# Autodesk Inventor assembly: Omniscope_new_v0
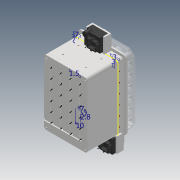
[picture p0: Inventor's stored thumbnail of the model, 180x180]
Saved by Autodesk Inventor 2022 (Build 260153000, 153)
## iProperties
Created: 2022-05-25
Part Number: Omniscope_new_v0
Document SubType Name: Assembly
Designer: diederichbenedict
Author: diederichbenedict
## Documents named in this file (13)
- C:\Users\diederichbenedict\Dropbox\Dokumente\Promotion\PROJECTS\Omniscope\INVENTOR\Omniscope_new_v0.iam
- C:\Users\diederichbenedict\Dropbox\Dokumente\Promotion\PROJECTS\Omniscope\INVENTOR\00_MicroSDCard.ipt
- C:\Users\diederichbenedict\Dropbox\Dokumente\Promotion\PROJECTS\Omniscope\INVENTOR\Omniscope_Base_v0.ipt
- C:\Users\diederichbenedict\Dropbox\Dokumente\Promotion\PROJECTS\Omniscope\INVENTOR\Omniscope_sidewalls_v0.ipt
- C:\Users\diederichbenedict\Dropbox\Dokumente\Promotion\PROJECTS\Omniscope\INVENTOR\Omniscope_mid_level_v0.ipt
- C:\Users\diederichbenedict\Dropbox\Dokumente\Promotion\PROJECTS\Omniscope\INVENTOR\OV_Camera.ipt
- C:\Users\diederichbenedict\Dropbox\Dokumente\Promotion\PROJECTS\Omniscope\INVENTOR\00_ESP3-CAMboard.iam
- C:\Users\diederichbenedict\Dropbox\Dokumente\Promotion\PROJECTS\Omniscope\INVENTOR\Omniscope_Camera_fix.ipt
- C:\Users\diederichbenedict\Dropbox\Dokumente\Promotion\PROJECTS\Omniscope\INVENTOR\00_24wellplate_base.ipt
- C:\Users\diederichbenedict\Dropbox\Dokumente\Promotion\PROJECTS\Omniscope\INVENTOR\Omniscope_sidewall_spacer_v0.ipt
- C:\Users\diederichbenedict\Dropbox\Dokumente\Promotion\PROJECTS\Omniscope\INVENTOR\Omniscope_lensmount_v0.ipt
- C:\Users\diederichbenedict\Dropbox\Dokumente\Promotion\PROJECTS\Omniscope\INVENTOR\00_Z_Focus_CCTV_Camera.ipt
- C:\Users\diederichbenedict\Dropbox\Dokumente\Promotion\PROJECTS\Omniscope\INVENTOR\Omniscope_Wellcarrier.ipt
## Components (106 placed, 12 different names)
1. Omniscope_Base_v0:1 — Passend:1, Passend:2, Passend:3, Fluchtend:3, Fluchtend:4
2. Omniscope_sidewalls_v0:1 — Fluchtend:3, Fluchtend:4, Einfügen:1, Einfügen:2, Passend:7, Fluchtend:7, Fluchtend:8, Fluchtend:15, Fluchtend:16, Passend:8, Passend:9, Passend:10, Fluchtend:17
3. Omniscope_mid_level_v0:1 — Einfügen:1, Einfügen:2, Passend:4, Winkel:1, Passend:5, Passend:6, Fluchtend:5, Fluchtend:6, Fluchtend:9
4. 00_24wellplate_base:1 — Passend:7, Fluchtend:7
5. Omniscope_sidewall_spacer_v0:1 — Fluchtend:8, Fluchtend:9, Fluchtend:10, Fluchtend:11
6. Omniscope_lensmount_v0:1 — Fluchtend:10, Fluchtend:11, Fluchtend:18, Fluchtend:19, Fluchtend:20
7. 00_Z_Focus_CCTV_Camera:1 — Fluchtend:13, Fluchtend:14, Fluchtend:15, Passend:9
8. 00_Z_Focus_CCTV_Camera:2 — Fluchtend:14, Fluchtend:16, Passend:8, Fluchtend:18
9. 00_Z_Focus_CCTV_Camera:3 — Fluchtend:13, Passend:10, Fluchtend:17
10. Omniscope_Wellcarrier:1 — Fluchtend:19, Fluchtend:20
11. 00_MicroSDCard:1 — Passend:1, Passend:2, Fluchtend:1, Fluchtend:2
12. 00_ESP3-CAMboard:1 — Fluchtend:1, Fluchtend:2, Passend:3
13. 00_MicroSDCard:2
14. 00_ESP3-CAMboard:2
15. 00_MicroSDCard:3
16. 00_ESP3-CAMboard:3
17. 00_MicroSDCard:4
18. 00_ESP3-CAMboard:4
19. 00_MicroSDCard:5
20. 00_ESP3-CAMboard:5
21. 00_MicroSDCard:6
22. 00_ESP3-CAMboard:6
23. 00_MicroSDCard:7
24. 00_ESP3-CAMboard:7
25. 00_MicroSDCard:8
26. 00_ESP3-CAMboard:8
27. 00_MicroSDCard:9
28. 00_ESP3-CAMboard:9
29. 00_MicroSDCard:10
30. 00_ESP3-CAMboard:10
31. 00_MicroSDCard:11
32. 00_ESP3-CAMboard:11
33. 00_MicroSDCard:12
34. 00_ESP3-CAMboard:12
35. 00_MicroSDCard:13
36. 00_ESP3-CAMboard:13
37. 00_MicroSDCard:14
38. 00_ESP3-CAMboard:14
39. 00_MicroSDCard:15
40. 00_ESP3-CAMboard:15
41. 00_MicroSDCard:16
42. 00_ESP3-CAMboard:16
43. 00_MicroSDCard:17
44. 00_ESP3-CAMboard:17
45. 00_MicroSDCard:18
46. 00_ESP3-CAMboard:18
47. 00_MicroSDCard:19
48. 00_ESP3-CAMboard:19
49. 00_MicroSDCard:20
50. 00_ESP3-CAMboard:20
51. 00_MicroSDCard:21
52. 00_ESP3-CAMboard:21
53. 00_MicroSDCard:22
54. 00_ESP3-CAMboard:22
55. 00_MicroSDCard:23
56. 00_ESP3-CAMboard:23
57. 00_MicroSDCard:24
58. 00_ESP3-CAMboard:24
59. Omniscope_Camera_fix:1 — Fluchtend:5, Fluchtend:6
60. OV_Camera:1 — Passend:4, Winkel:1, Passend:5, Passend:6
61. Omniscope_Camera_fix:2
62. OV_Camera:2
63. Omniscope_Camera_fix:3
64. OV_Camera:3
65. Omniscope_Camera_fix:4
66. OV_Camera:4
67. Omniscope_Camera_fix:5
68. OV_Camera:5
69. Omniscope_Camera_fix:6
70. OV_Camera:6
71. Omniscope_Camera_fix:7
72. OV_Camera:7
73. Omniscope_Camera_fix:8
74. OV_Camera:8
75. Omniscope_Camera_fix:9
76. OV_Camera:9
77. Omniscope_Camera_fix:10
78. OV_Camera:10
79. Omniscope_Camera_fix:11
80. OV_Camera:11
81. Omniscope_Camera_fix:12
82. OV_Camera:12
83. Omniscope_Camera_fix:13
84. OV_Camera:13
85. Omniscope_Camera_fix:14
86. OV_Camera:14
87. Omniscope_Camera_fix:15
88. OV_Camera:15
89. Omniscope_Camera_fix:16
90. OV_Camera:16
91. Omniscope_Camera_fix:17
92. OV_Camera:17
93. Omniscope_Camera_fix:18
94. OV_Camera:18
95. Omniscope_Camera_fix:19
96. OV_Camera:19
97. Omniscope_Camera_fix:20
98. OV_Camera:20
99. Omniscope_Camera_fix:21
100. OV_Camera:21
101. Omniscope_Camera_fix:22
102. OV_Camera:22
103. Omniscope_Camera_fix:23
104. OV_Camera:23
105. Omniscope_Camera_fix:24
106. OV_Camera:24
## Component patterns: (24 elements, first: 00_MicroSDCard:1 + 00_ESP3-CAMboard:1), (24 elements, first: Omniscope_Camera_fix:1 + OV_Camera:1)
## Relationships (32: Flush 19, Mate 10, Insert 2, Angle 1)
- Passend:1 [Mate]: Omniscope_Base_v0:1 ↔ 00_MicroSDCard:1
- Passend:2 [Mate]: Omniscope_Base_v0:1 ↔ 00_MicroSDCard:1
- Fluchtend:1 [Flush]: 00_MicroSDCard:1 ↔ 00_ESP3-CAMboard:1
- Fluchtend:2 [Flush]: 00_MicroSDCard:1 ↔ 00_ESP3-CAMboard:1
- Passend:3 [Mate] (14 mm): Omniscope_Base_v0:1 ↔ 00_ESP3-CAMboard:1
- Fluchtend:3 [Flush]: Omniscope_Base_v0:1 ↔ Omniscope_sidewalls_v0:1
- Fluchtend:4 [Flush]: Omniscope_Base_v0:1 ↔ Omniscope_sidewalls_v0:1
- Einfügen:1 [Insert]: Omniscope_sidewalls_v0:1 ↔ Omniscope_mid_level_v0:1
- Einfügen:2 [Insert]: Omniscope_sidewalls_v0:1 ↔ Omniscope_mid_level_v0:1
- Passend:4 [Mate] (-1 mm): Omniscope_mid_level_v0:1 ↔ OV_Camera:1
- Winkel:1 [Angle] (0 deg): Omniscope_mid_level_v0:1 ↔ OV_Camera:1
- Passend:5 [Mate] (0.2 mm): Omniscope_mid_level_v0:1 ↔ OV_Camera:1
- Passend:6 [Mate]: Omniscope_mid_level_v0:1 ↔ OV_Camera:1
- Fluchtend:5 [Flush]: Omniscope_mid_level_v0:1 ↔ Omniscope_Camera_fix:1
- Fluchtend:6 [Flush] (2 mm): Omniscope_mid_level_v0:1 ↔ Omniscope_Camera_fix:1
- Passend:7 [Mate]: Omniscope_sidewalls_v0:1 ↔ 00_24wellplate_base:1
- Fluchtend:7 [Flush]: Omniscope_sidewalls_v0:1 ↔ 00_24wellplate_base:1
- Fluchtend:8 [Flush]: Omniscope_sidewalls_v0:1 ↔ Omniscope_sidewall_spacer_v0:1
- Fluchtend:9 [Flush]: Omniscope_mid_level_v0:1 ↔ Omniscope_sidewall_spacer_v0:1
- Fluchtend:10 [Flush]: Omniscope_sidewall_spacer_v0:1 ↔ Omniscope_lensmount_v0:1
- Fluchtend:11 [Flush]: Omniscope_sidewall_spacer_v0:1 ↔ Omniscope_lensmount_v0:1
- Fluchtend:13 [Flush]: 00_Z_Focus_CCTV_Camera:1 ↔ 00_Z_Focus_CCTV_Camera:3
- Fluchtend:14 [Flush]: 00_Z_Focus_CCTV_Camera:1 ↔ 00_Z_Focus_CCTV_Camera:2
- Fluchtend:15 [Flush] (3 mm): Omniscope_sidewalls_v0:1 ↔ 00_Z_Focus_CCTV_Camera:1
- Fluchtend:16 [Flush] (3 mm): Omniscope_sidewalls_v0:1 ↔ 00_Z_Focus_CCTV_Camera:2
- Passend:8 [Mate] (3 mm): Omniscope_sidewalls_v0:1 ↔ 00_Z_Focus_CCTV_Camera:2
- Passend:9 [Mate] (3 mm): Omniscope_sidewalls_v0:1 ↔ 00_Z_Focus_CCTV_Camera:1
- Passend:10 [Mate] (3 mm): Omniscope_sidewalls_v0:1 ↔ 00_Z_Focus_CCTV_Camera:3
- Fluchtend:17 [Flush]: Omniscope_sidewalls_v0:1 ↔ 00_Z_Focus_CCTV_Camera:3
- Fluchtend:18 [Flush] (3 mm): Omniscope_lensmount_v0:1 ↔ 00_Z_Focus_CCTV_Camera:2
- Fluchtend:19 [Flush]: Omniscope_lensmount_v0:1 ↔ Omniscope_Wellcarrier:1
- Fluchtend:20 [Flush]: Omniscope_lensmount_v0:1 ↔ Omniscope_Wellcarrier:1
